# Autodesk Inventor assembly: largeCapAssemblyGlued
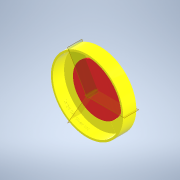
[picture p0: Inventor's stored thumbnail of the model, 180x180]
Saved by Autodesk Inventor 2021.1 (Build 251245010, 245A)
## iProperties
Created: 2020-09-25
Part Number: largeCapAssemblyGlued
Document SubType Name: Assembly
Designer: robst
Author: robst
## Documents named in this file (3)
- C:\git\CAD-Development\robSteele\HouseProjects\Garage\CapForWater\largeCapAssemblyGlued.iam
- C:\git\CAD-Development\robSteele\HouseProjects\Garage\CapForWater\largeCap.ipt
- C:\git\CAD-Development\robSteele\HouseProjects\Garage\CapForWater\supportRingsForLargeCap.ipt
## Components (4 placed, 2 different names)
1. supportRingsForLargeCap:1 — Mate:1, Insert:1
2. largeCap:1 — Mate:1, Insert:1
3. largeCap:2
4. largeCap:3
## Component patterns: (3 elements, first: largeCap:1)
## Relationships (2: Mate 1, Insert 1)
- Mate:1: supportRingsForLargeCap:1 ↔ largeCap:1
- Insert:1: supportRingsForLargeCap:1 ↔ largeCap:1
